# Autodesk Inventor assembly: Fan+Bracket
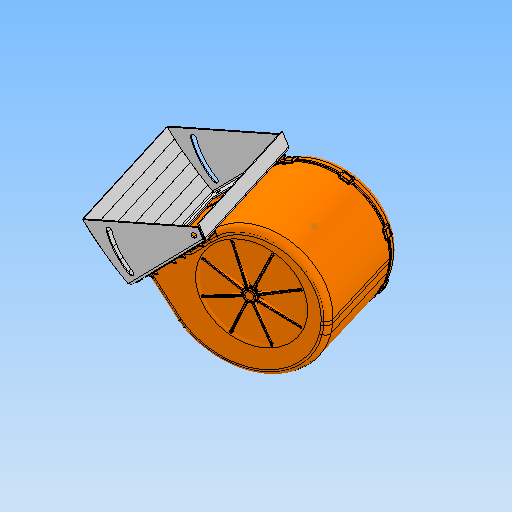
[picture p0: Inventor's stored thumbnail of the model, 512x512]
Saved by Autodesk Inventor 2025.4 (Build 294407000, 407)
## iProperties
Created: 2025-10-21
Part Number: Fan+Bracket
Document SubType Name: Assembly
Designer: josh
Author: josh
## Documents named in this file (3)
- R:\A1- Neuweg Design Data\OM Robotics\CLEANING BRUSH CAGE & ROLLER\Fan+Bracket.iam
- R:\A1- Neuweg Design Data\OM Robotics\CLEANING BRUSH CAGE & ROLLER\Fan Bracket.ipt
- R:\A1- Neuweg Design Data\OM Robotics\CLEANING BRUSH CAGE & ROLLER\007-B42-32D.ipt
## Components (2 placed, 2 different names)
1. Fan Bracket:1
2. 007-B42-32D:1
## Relationships (1: Insert 1)
- [Insert]: Fan Bracket:1 ↔ 007-B42-32D:1
